# Autodesk Inventor assembly: HopperSupportAssembly
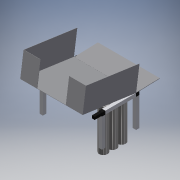
[picture p0: Inventor's stored thumbnail of the model, 180x180]
Saved by Autodesk Inventor 2017 (Build 210142000, 142)
## iProperties
Created: 2020-02-22
Part Number: HopperSupportAssembly
Document SubType Name: Assembly
Designer: S338674153
Author: S338674153
## Documents named in this file (9)
- \\ad.ocdsb.ca\studenthome\3\S338674153\FRC 2020\FullRobotRefactor\Hopper\HopperSupportAssembly.iam
- \\ad.ocdsb.ca\studenthome\3\S338674153\FRC 2020\FullRobotRefactor\Hopper\HopperSupport.ipt
- \\ad.ocdsb.ca\studenthome\3\S338674153\FRC 2020\FullRobotRefactor\Hopper\1in sq tub - 10-875.ipt
- \\ad.ocdsb.ca\studenthome\3\S338674153\FRC 2020\FullRobotRefactor\KIPS\Kipp K0617.ipt
- \\ad.ocdsb.ca\studenthome\3\S338674153\FRC 2020\FullRobotRefactor\Hopper\1in sq tub - 16-5.ipt
- \\ad.ocdsb.ca\studenthome\3\S338674153\FRC 2020\FullRobotRefactor\KIPS\Kipp K0619.ipt
- \\ad.ocdsb.ca\studenthome\3\S338674153\FRC 2020\FullRobotRefactor\Hopper\hopper_bottom2.ipt
- \\ad.ocdsb.ca\studenthome\3\S338674153\FRC 2020\FullRobotRefactor\Hopper\HopperWall.ipt
- \\ad.ocdsb.ca\studenthome\3\S338674153\FRC 2020\FullRobotRefactor\Parts\AirTank.ipt
## Components (16 placed, 8 different names)
1. HopperSupport:2 — Mate:12, Mate:13, Mate:14
2. HopperSupport:3 — Mate:3, Mate:4, Mate:5
3. HopperSupport:4 — Mate:18, Mate:19, Mate:20
4. 1in sq tub - 10-875:1 — Flush:4, Mate:21, Mate:22, Mate:23, Flush:5, Mate:24, Flush:6, Angle:1
5. 1in sq tub - 10-875:2 — Mate:1, Flush:2, Flush:3, Mate:2, Mate:6, Mate:7, Mate:8, Tangent:2, Tangent:3, Tangent:4
6. Kipp K0617:2 — Mate:1, Flush:2, Flush:3, Mate:2, Mate:3, Mate:4, Mate:5
7. 1in sq tub - 16-5:1 — Mate:9, Mate:10, Mate:11, Mate:15, Mate:16, Mate:17, Mate:28
8. Kipp K0619:1 — Mate:6, Mate:7, Mate:8, Mate:9, Mate:10, Mate:11, Mate:12, Mate:13, Mate:14
9. HopperSupport:5 — Mate:25, Mate:26, Mate:27
10. Kipp K0619:2 — Mate:15, Mate:16, Mate:17, Mate:18, Mate:19, Mate:20, Flush:4, Mate:21, Mate:22
11. Kipp K0617:3 — Mate:23, Flush:5, Mate:24, Mate:25, Mate:26, Mate:27
12. hopper_bottom2:1 — Flush:6, Mate:28, Angle:1, Mate:29, Flush:7, Angle:2
13. HopperWall:1 — Mate:29, Flush:7, Angle:2
14. AirTank:1 — Tangent:4
15. AirTank:2 — Tangent:2
16. AirTank:3 — Tangent:3
## Relationships (40: Mate 29, Flush 6, Tangent 3, Angle 2)
- Mate:1: 1in sq tub - 10-875:2 ↔ Kipp K0617:2
- Flush:2: 1in sq tub - 10-875:2 ↔ Kipp K0617:2
- Flush:3: 1in sq tub - 10-875:2 ↔ Kipp K0617:2
- Mate:2: 1in sq tub - 10-875:2 ↔ Kipp K0617:2
- Mate:3: HopperSupport:3 ↔ Kipp K0617:2
- Mate:4: HopperSupport:3 ↔ Kipp K0617:2
- Mate:5: HopperSupport:3 ↔ Kipp K0617:2
- Mate:6: 1in sq tub - 10-875:2 ↔ Kipp K0619:1
- Mate:7: 1in sq tub - 10-875:2 ↔ Kipp K0619:1
- Mate:8: 1in sq tub - 10-875:2 ↔ Kipp K0619:1
- Mate:9: 1in sq tub - 16-5:1 ↔ Kipp K0619:1
- Mate:10: 1in sq tub - 16-5:1 ↔ Kipp K0619:1
- Mate:11: 1in sq tub - 16-5:1 ↔ Kipp K0619:1
- Mate:12: HopperSupport:2 ↔ Kipp K0619:1
- Mate:13: HopperSupport:2 ↔ Kipp K0619:1
- Mate:14: HopperSupport:2 ↔ Kipp K0619:1
- Mate:15: 1in sq tub - 16-5:1 ↔ Kipp K0619:2
- Mate:16: 1in sq tub - 16-5:1 ↔ Kipp K0619:2
- Mate:17: 1in sq tub - 16-5:1 ↔ Kipp K0619:2
- Mate:18: HopperSupport:4 ↔ Kipp K0619:2
- Mate:19: HopperSupport:4 ↔ Kipp K0619:2
- Mate:20: HopperSupport:4 ↔ Kipp K0619:2
- Flush:4: 1in sq tub - 10-875:1 ↔ Kipp K0619:2
- Mate:21: 1in sq tub - 10-875:1 ↔ Kipp K0619:2
- Mate:22: 1in sq tub - 10-875:1 ↔ Kipp K0619:2
- Mate:23: 1in sq tub - 10-875:1 ↔ Kipp K0617:3
- Flush:5: 1in sq tub - 10-875:1 ↔ Kipp K0617:3
- Mate:24: 1in sq tub - 10-875:1 ↔ Kipp K0617:3
- Mate:25: HopperSupport:5 ↔ Kipp K0617:3
- Mate:26: HopperSupport:5 ↔ Kipp K0617:3
- Mate:27: HopperSupport:5 ↔ Kipp K0617:3
- Flush:6: 1in sq tub - 10-875:1 ↔ hopper_bottom2:1
- Mate:28: 1in sq tub - 16-5:1 ↔ hopper_bottom2:1
- Angle:1 (188.1 deg): 1in sq tub - 10-875:1 ↔ hopper_bottom2:1
- Mate:29: hopper_bottom2:1 ↔ HopperWall:1
- Flush:7: hopper_bottom2:1 ↔ HopperWall:1
- Angle:2 (180 deg): hopper_bottom2:1 ↔ HopperWall:1
- Tangent:2: 1in sq tub - 10-875:2 ↔ AirTank:2
- Tangent:3: 1in sq tub - 10-875:2 ↔ AirTank:3
- Tangent:4: 1in sq tub - 10-875:2 ↔ AirTank:1
